# Autodesk Inventor assembly: assembly all
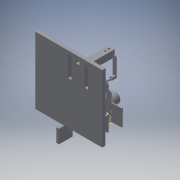
[picture p0: Inventor's stored thumbnail of the model, 180x180]
Saved by Autodesk Inventor 2019 (Build 230136000, 136)
## iProperties
Created: 2020-03-01
Part Number: assembly all
Document SubType Name: Assembly
Designer: VIGNESH
Author: VIGNESH
## Documents named in this file (15)
- C:\Users\VIGNESH\Documents\assembly all.iam
- C:\Users\VIGNESH\Documents\Part4.ipt
- C:\Users\VIGNESH\Documents\big servo.ipt
- C:\Users\VIGNESH\Documents\base 3.ipt
- C:\Users\VIGNESH\Documents\base 4.ipt
- C:\Users\VIGNESH\Documents\motor 2.ipt
- C:\Users\VIGNESH\Documents\base 5.ipt
- C:\Users\VIGNESH\Documents\load cell.ipt
- C:\Users\VIGNESH\Documents\motor wing.ipt
- C:\Users\VIGNESH\Documents\load stand.ipt
- C:\Users\VIGNESH\Documents\5 mm bolt.ipt
- C:\Users\VIGNESH\Documents\5mm fixer.ipt
- C:\Users\VIGNESH\Documents\5mm l=10mm.ipt
- C:\Users\VIGNESH\Documents\now 2.iam
- C:\Users\VIGNESH\Documents\5mm bolt 40 mm height.ipt
## Components (23 placed, 14 different names)
1. Part4:1 — Mate:1, Mate:2, Mate:3, Mate:4, Mate:5, Mate:7
2. big servo:1 — Mate:1
3. base 3:1 — Mate:2
4. base 3:2 — Mate:3
5. base 4:1 — Mate:5
6. base 4:2 — Mate:4
7. motor 2:1 — Rotational:1
8. base 5:1
9. load cell:1 — Mate:7, Mate:8, Mate:9, Mate:10, Rotational:2
10. motor wing:1 — Rotational:1
11. load stand:1 — Mate:8, Mate:9, Mate:10, Rotational:3, Rotational:6
12. load stand:2 — Rotational:7
13. 5 mm bolt:1 — Rotational:3, Rotational:5
14. 5 mm bolt:2 — Rotational:2, Rotational:4
15. 5mm fixer:2 — Rotational:5
16. 5mm fixer:3 — Rotational:4
17. 5mm l=10mm:1 — Rotational:7
18. 5mm l=10mm:2 — Rotational:6
19. now 2:1 [sub-assembly]
20. 5mm bolt 40 mm height:1
21. 5mm bolt 40 mm height:2
22. 5mm bolt 40 mm height:3
23. 5mm bolt 40 mm height:4
## Relationships (16: Mate 9, RevoluteJoint 7)
- Mate:1: Part4:1 ↔ big servo:1
- Mate:2: Part4:1 ↔ base 3:1
- Mate:3: Part4:1 ↔ base 3:2
- Mate:4: Part4:1 ↔ base 4:2
- Mate:5: Part4:1 ↔ base 4:1
- Mate:7: Part4:1 ↔ load cell:1
- Rotational:1 [RevoluteJoint] (-6 mm): motor 2:1 ↔ motor wing:1
- Mate:8: load cell:1 ↔ load stand:1
- Mate:9: load cell:1 ↔ load stand:1
- Mate:10: load cell:1 ↔ load stand:1
- Rotational:2 [RevoluteJoint] (25 mm): load cell:1 ↔ 5 mm bolt:2
- Rotational:3 [RevoluteJoint] (-25 mm): load stand:1 ↔ 5 mm bolt:1
- Rotational:4 [RevoluteJoint] (5 mm): 5 mm bolt:2 ↔ 5mm fixer:3
- Rotational:5 [RevoluteJoint] (-2 mm): 5 mm bolt:1 ↔ 5mm fixer:2
- Rotational:6 [RevoluteJoint] (10 mm): load stand:1 ↔ 5mm l=10mm:2
- Rotational:7 [RevoluteJoint] (10 mm): load stand:2 ↔ 5mm l=10mm:1
